# Autodesk Inventor assembly: 412
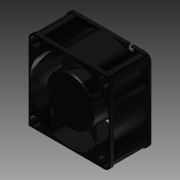
[picture p0: Inventor's stored thumbnail of the model, 180x180]
Saved by Autodesk Inventor 2013 (Build 170138000, 138)
## iProperties
Category: Electrical
Company: Autodesk Inc.
Shininess: 64.0
Length Units: 11272
Angle Units: 11279
Time Units: 11290
Mass Units: 11286
Length Display Precision: 3
Angle Display Precision: 2
Compacted: True
Part Number: 412
Document SubType Name: Assembly
Created: 2012-11-26
Designer: Autodesk Inc.
Description: Comapct fan - mini 12V DC
Catalog Web Link: http://www.ebmpapst.us/allpdfs/400.PDF
Vendor: ebmpapst
Density: 0.0
Volumn: 0.0
Area: 0.0
PropertySet Name: Model Information
Control State: 0
Master: False
Checked Out: False
Author: Autodesk Inc.
## Documents named in this file (3)
- C:\Users\Arpan\Documents\GitHub\frc2013CAD\Electrical\ELEC_FanMini_412.iam
- C:\Users\Arpan\Documents\GitHub\frc2013CAD\Electrical\fan body.ipt
- C:\Users\Arpan\Documents\GitHub\frc2013CAD\Electrical\fan blade.ipt
## Components (2 placed, 2 different names)
1. fan body:1 — Flush:1, Mate:1
2. fan blade:1 — Flush:1, Mate:1
## Relationships (2: Flush 1, Mate 1)
- Flush:1: fan body:1 ↔ fan blade:1
- Mate:1: fan body:1 ↔ fan blade:1
